# Autodesk Inventor assembly: RightMecanum-SubAssem01
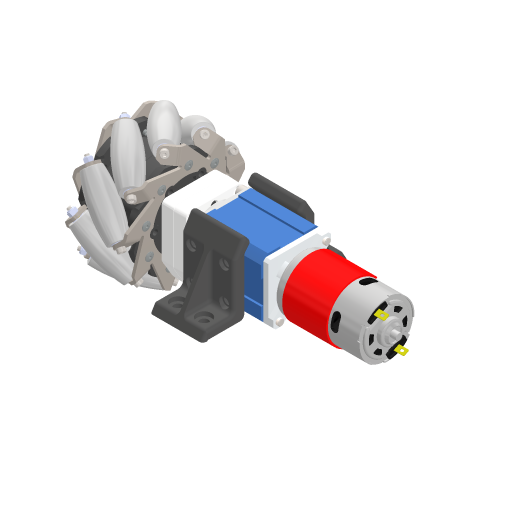
[picture p0: Inventor's stored thumbnail of the model, 512x512]
Saved by Autodesk Inventor 2024 (Build 280153000, 153)
## iProperties
Created: 2022-07-11
Part Number: RightMecanum-SubAssem01
Document SubType Name: Assembly
Designer: Dave
Author: Dave
## Documents named in this file (9)
- C:\Autodesk\ChalkBot Github\ChalkbotMechanical\Chalkbot1.0\Chassis\V1\RightMecanum-SubAssem01.iam
- C:\Autodesk\ChalkBot Github\ChalkbotMechanical\Chalkbot1.0\Chassis\V1\Mechanum STEP files\am-3775a AndyMark RedLine Motor (1).ipt
- C:\Autodesk\ChalkBot Github\ChalkbotMechanical\Chalkbot1.0\Chassis\V1\Motor and Gearbox STEP files\Hex Bore Mag Encoder Housing (217-6785).iam
- C:\Autodesk\ChalkBot Github\ChalkbotMechanical\Chalkbot1.0\Chassis\V1\Motor and Gearbox STEP files\am-3791 - 3000 x 500 Hex Shaft.ipt
- C:\Autodesk\ChalkBot Github\ChalkbotMechanical\Chalkbot1.0\Chassis\V1\Motor and Gearbox STEP files\2 Stage HD - 57 Sport.ipt
- C:\Autodesk\ChalkBot Github\ChalkbotMechanical\Chalkbot1.0\Chassis\V1\Motor Mounts.ipt
- C:\Autodesk\ChalkBot Github\ChalkbotMechanical\Chalkbot1.0\Chassis\V1\Shaft Spacers V2.ipt
- C:\Autodesk\ChalkBot Github\ChalkbotMechanical\Chalkbot1.0\Chassis\V1\Mechanum STEP files\am-3918L 4HD 500H Mecanum Right.iam
- C:\Autodesk\ChalkBot Github\ChalkbotMechanical\Chalkbot1.0\Chassis\V1\Motor and Gearbox STEP files\am-2986 FR8ZZ Hex Bearing.ipt
## Components (15 placed, 8 different names)
1. 2 Stage HD - 57 Sport:1 — Insert:4, Angle:1, Insert:6, Insert:7, Insert:8, Insert:9, Rotational:1, Cylindrical:1, Rigid:2
2. am-3775a AndyMark RedLine Motor (1):1 — Rigid:2
3. Hex Bore Mag Encoder Housing (217-6785):1 [sub-assembly] — Rotational:1, Cylindrical:1, Mate:4
4. am-3791 - 3000 x 500 Hex Shaft:1 — Insert:4, Mate:5, Mate:6, Mate:8, Mate:9, Mate:11, Mate:12
5. Motor Mounts:1 — Insert:6, Insert:7
6. Motor Mounts:2 — Insert:8, Insert:9
7. Shaft Spacers V2:1 — Rigid:3, Rigid:4
8. Shaft Spacers V2:2 — Rigid:3, Rigid:5
9. Shaft Spacers V2:3 — Rigid:4, Rigid:6
10. Shaft Spacers V2:4 — Rigid:5, Rigid:7
11. Shaft Spacers V2:5 — Rigid:6, Mate:4
12. Shaft Spacers V2:6 — Rigid:7, Rigid:8
13. Shaft Spacers V2:7 — Rigid:8, Mate:5, Mate:6, Mate:7
14. am-3918L 4HD 500H Mecanum Right:1 [sub-assembly] — Mate:7, Mate:8, Mate:9, Mate:10
15. am-2986 FR8ZZ Hex Bearing:1 — Mate:10, Mate:11, Mate:12
## Relationships (25: Mate 9, WeldJoint 7, Insert 6, Angle 1, RevoluteJoint 1, CylindricalJoint 1)
- [Insert]: 2 Stage HD - 57 Sport:1 ↔ am-3791 - 3000 x 500 Hex Shaft:1
- Insert:4: 2 Stage HD - 57 Sport:1 ↔ am-3791 - 3000 x 500 Hex Shaft:1
- Angle:1 (0 deg): 2 Stage HD - 57 Sport:1
- Insert:6: 2 Stage HD - 57 Sport:1 ↔ Motor Mounts:1
- Insert:7: 2 Stage HD - 57 Sport:1 ↔ Motor Mounts:1
- Insert:8: 2 Stage HD - 57 Sport:1 ↔ Motor Mounts:2
- Insert:9: 2 Stage HD - 57 Sport:1 ↔ Motor Mounts:2
- Rotational:1 [RevoluteJoint]: 2 Stage HD - 57 Sport:1 ↔ Hex Bore Mag Encoder Housing (217-6785):1
- Cylindrical:1: 2 Stage HD - 57 Sport:1 ↔ Hex Bore Mag Encoder Housing (217-6785):1
- Rigid:2 [WeldJoint]: 2 Stage HD - 57 Sport:1 ↔ am-3775a AndyMark RedLine Motor (1):1
- Rigid:3 [WeldJoint]: Shaft Spacers V2:1 ↔ Shaft Spacers V2:2
- Rigid:4 [WeldJoint]: Shaft Spacers V2:1 ↔ Shaft Spacers V2:3
- Rigid:5 [WeldJoint]: Shaft Spacers V2:2 ↔ Shaft Spacers V2:4
- Rigid:6 [WeldJoint]: Shaft Spacers V2:3 ↔ Shaft Spacers V2:5
- Rigid:7 [WeldJoint]: Shaft Spacers V2:4 ↔ Shaft Spacers V2:6
- Rigid:8 [WeldJoint]: Shaft Spacers V2:6 ↔ Shaft Spacers V2:7
- Mate:4: Hex Bore Mag Encoder Housing (217-6785):1 ↔ Shaft Spacers V2:5
- Mate:5 (0.15 mm): am-3791 - 3000 x 500 Hex Shaft:1 ↔ Shaft Spacers V2:7
- Mate:6 (0.15 mm): am-3791 - 3000 x 500 Hex Shaft:1 ↔ Shaft Spacers V2:7
- Mate:7: Shaft Spacers V2:7 ↔ am-3918L 4HD 500H Mecanum Right:1
- Mate:8: am-3791 - 3000 x 500 Hex Shaft:1 ↔ am-3918L 4HD 500H Mecanum Right:1
- Mate:9: am-3791 - 3000 x 500 Hex Shaft:1 ↔ am-3918L 4HD 500H Mecanum Right:1
- Mate:10: am-3918L 4HD 500H Mecanum Right:1 ↔ am-2986 FR8ZZ Hex Bearing:1
- Mate:11: am-3791 - 3000 x 500 Hex Shaft:1 ↔ am-2986 FR8ZZ Hex Bearing:1
- Mate:12: am-3791 - 3000 x 500 Hex Shaft:1 ↔ am-2986 FR8ZZ Hex Bearing:1
